# Autodesk Inventor assembly: Ensamblaje1
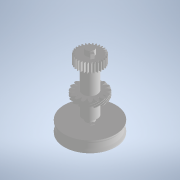
[picture p0: Inventor's stored thumbnail of the model, 180x180]
Saved by Autodesk Inventor 2022 (Build 260153000, 153)
## iProperties
Created: 2024-04-07
Part Number: Ensamblaje1
Document SubType Name: Assembly
Designer: Lourdes Ac Minera
Author: Lourdes Ac Minera
## Documents named in this file (6)
- C:\Users\Lourdes Ac Minera\Documents\7 SEMESTRE\Dinámica\Lab\Tarea 4 - Ensamble\Ensamblaje1.iam
- C:\Users\Lourdes Ac Minera\Documents\7 SEMESTRE\Dinámica\Lab\Tarea 4 - Ensamble\Eje cuñero.ipt
- C:\Users\Lourdes Ac Minera\Documents\7 SEMESTRE\Dinámica\Lab\Tarea 4 - Ensamble\Cuña.ipt
- C:\Users\Lourdes Ac Minera\Documents\7 SEMESTRE\Dinámica\Lab\Tarea 4 - Ensamble\Engranaje.ipt
- C:\Users\Lourdes Ac Minera\Documents\7 SEMESTRE\Dinámica\Lab\Tarea 4 - Ensamble\Polea.ipt
- C:\Users\Lourdes Ac Minera\Documents\7 SEMESTRE\Dinámica\Lab\Tarea 4 - Ensamble\Engrane helicoidal.ipt
## Components (6 placed, 5 different names)
1. Eje cuñero:1 — Rígido:1, Rígido:2, Coincidencia:1, Coincidencia:2, Cilíndrica:1, Coincidencia:5
2. Cuña:1 — Rígido:1, Coincidencia:3
3. Cuña:2 — Rígido:2, Coincidencia:4
4. Engranaje:1 — Coincidencia:1, Coincidencia:4
5. Polea:1 — Coincidencia:2, Coincidencia:3, Coincidencia:5
6. Engrane helicoidal:2 — Cilíndrica:1
## Relationships (8: Mate 5, WeldJoint 2, CylindricalJoint 1)
- Rígido:1 [WeldJoint]: Eje cuñero:1 ↔ Cuña:1
- Rígido:2 [WeldJoint]: Eje cuñero:1 ↔ Cuña:2
- Coincidencia:1 [Mate]: Eje cuñero:1 ↔ Engranaje:1
- Coincidencia:2 [Mate]: Eje cuñero:1 ↔ Polea:1
- Coincidencia:3 [Mate]: Cuña:1 ↔ Polea:1
- Coincidencia:4 [Mate]: Cuña:2 ↔ Engranaje:1
- Cilíndrica:1 [CylindricalJoint]: Eje cuñero:1 ↔ Engrane helicoidal:2
- Coincidencia:5 [Mate]: Eje cuñero:1 ↔ Polea:1
